# Autodesk Inventor assembly: bot
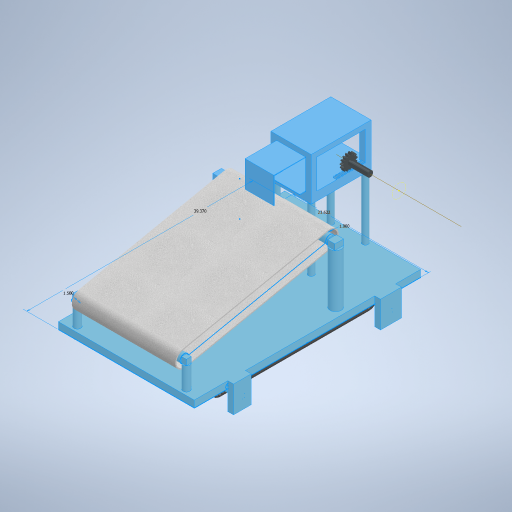
[picture p0: Inventor's stored thumbnail of the model, 512x512]
Saved by Autodesk Inventor 2024 (Build 280153000, 153)
## iProperties
Created: 2023-06-13
Part Number: bot
Document SubType Name: Assembly
Designer: rajen
Author: rajen
## Documents named in this file (5)
- C:\Users\Hp\Desktop\BOT\bot.iam
- C:\Users\Hp\Desktop\BOT\gear_neha.ipt
- C:\Users\Hp\Desktop\BOT\neha_chassis (1).ipt
- C:\Users\Hp\Desktop\BOT\bult.ipt
- C:\Users\Hp\Desktop\BOT\gear fzfger.ipt
## Components (6 placed, 4 different names)
1. gear_neha:1 — Rigid:2
2. gear_neha:2 — Rigid:1, Rotational:1
3. neha_chassis (1):2 — Rigid:1, Rigid:2, Rotational:2, Rigid:3
4. bult:1 — Rotational:2
5. bult:2 — Rotational:1
6. gear fzfger:1 — Rigid:3
## Relationships (5: WeldJoint 3, RevoluteJoint 2)
- Rigid:1 [WeldJoint]: gear_neha:2 ↔ neha_chassis (1):2
- Rigid:2 [WeldJoint]: gear_neha:1 ↔ neha_chassis (1):2
- Rotational:1 [RevoluteJoint]: gear_neha:2 ↔ bult:2
- Rotational:2 [RevoluteJoint]: neha_chassis (1):2 ↔ bult:1
- Rigid:3 [WeldJoint]: neha_chassis (1):2 ↔ gear fzfger:1
